# Autodesk Inventor assembly: wheel_assembly
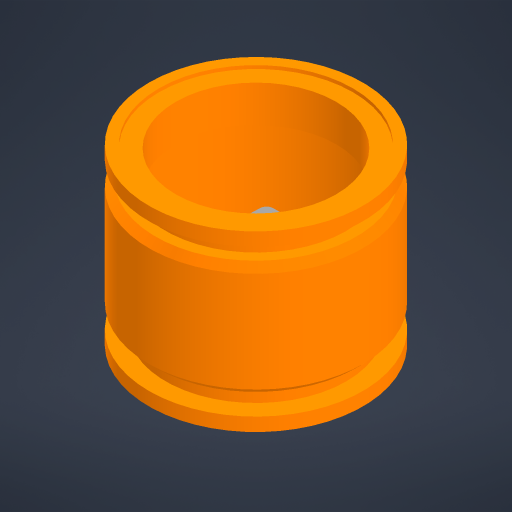
[picture p0: Inventor's stored thumbnail of the model, 512x512]
Saved by Autodesk Inventor 2024 (Build 280153000, 153)
## iProperties
Created: 2023-10-16
Part Number: wheel_assembly
Document SubType Name: Assembly
Designer: user
Author: user
## Documents named in this file (4)
- D:\Docs\Robot\3d_v2\machine_body\arm_assembly\wheel_assembly.iam
- D:\Docs\Robot\3d_v2\default_components\tire.ipt
- D:\Docs\Robot\3d_v2\machine_body\wheel_assembly\wheel.ipt
- D:\Docs\Robot\3d_v2\default_components\nohex.ipt
## Components (3 placed, 3 different names)
1. tire:1 — Совмещение:1, Совмещение:2, Совмещение:3, Вставка:1
2. wheel:1 — Вставка:1, Совмещение:4, Вставка:2
3. nohex:1 — Угол:1, Вставка:2
## Relationships (7: Mate 4, Insert 2, Angle 1)
- Совмещение:1 [Mate]: tire:1
- Совмещение:2 [Mate]: tire:1
- Совмещение:3 [Mate]: tire:1
- Вставка:1 [Insert]: tire:1 ↔ wheel:1
- Совмещение:4 [Mate]: wheel:1
- Угол:1 [Angle] (-2 deg): nohex:1
- Вставка:2 [Insert]: wheel:1 ↔ nohex:1
